# Autodesk Inventor assembly: SevoWithServoPlateActobotics
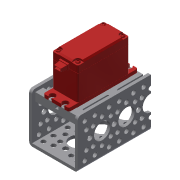
[picture p0: Inventor's stored thumbnail of the model, 180x180]
Saved by Autodesk Inventor 2018 (Build 220112000, 112)
## iProperties
Created: 2018-12-09
Part Number: SevoWithServoPlateActobotics
Document SubType Name: Assembly
Designer: ball
Author: ball
## Documents named in this file (4)
- C:\FTC\FTC8863CAD\2018Robot\SevoWithServoPlateActobotics.iam
- C:\FTC\FTC8863CAD\Actobotics\585 parts\Channel2Hole.ipt
- C:\FTC\FTC8863CAD\Actobotics\575 parts\575124.ipt
- C:\FTC\FTC8863CAD\GoBilda\2000 Parts\2000-0025-0001 part.ipt
## Components (3 placed, 3 different names)
1. Channel2Hole:1 — Mate:1, Mate:2, Mate:3, Mate:6, Angle:1
2. 575124:1 — Mate:1, Mate:2, Mate:3, Mate:5
3. 2000-0025-0001 part:1 — Mate:5, Mate:6, Angle:1
## Relationships (6: Mate 5, Angle 1)
- Mate:1: Channel2Hole:1 ↔ 575124:1
- Mate:2: Channel2Hole:1 ↔ 575124:1
- Mate:3: Channel2Hole:1 ↔ 575124:1
- Mate:5: 575124:1 ↔ 2000-0025-0001 part:1
- Mate:6: Channel2Hole:1 ↔ 2000-0025-0001 part:1
- Angle:1 (0 deg): Channel2Hole:1 ↔ 2000-0025-0001 part:1
